# Autodesk Inventor assembly: robot
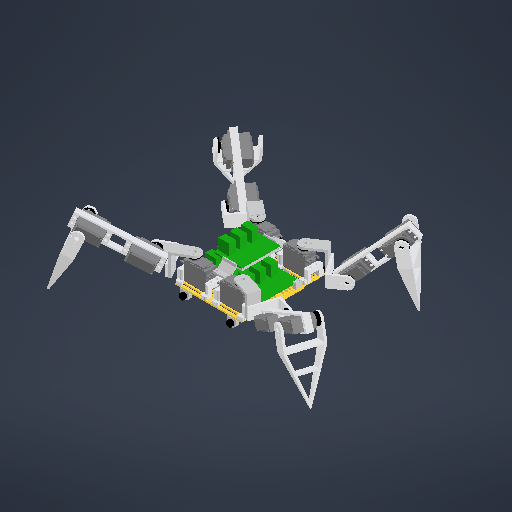
[picture p0: Inventor's stored thumbnail of the model, 512x512]
Saved by Autodesk Inventor 2026.1 (Build 301233000, 233)
## iProperties
Created: 2025-10-02
Part Number: robot
Document SubType Name: Assembly
Designer: emanuel
Author: emanuel
## Documents named in this file (16)
- C:\Users\emanuel\UnFolder\SpiderRobo\3dmodel\robot.iam
- C:\Users\emanuel\UnFolder\SpiderRobo\3dmodel\calf.ipt
- C:\Users\emanuel\UnFolder\SpiderRobo\3dmodel\femur.ipt
- C:\Users\emanuel\UnFolder\SpiderRobo\3dmodel\L1.ipt
- C:\Users\emanuel\UnFolder\SpiderRobo\3dmodel\L2.ipt
- C:\Users\emanuel\UnFolder\SpiderRobo\3dmodel\mg996r.ipt
- C:\Users\emanuel\UnFolder\SpiderRobo\3dmodel\prototype_pcb.ipt
- C:\Users\emanuel\UnFolder\SpiderRobo\3dmodel\servo_disc.ipt
- C:\Users\emanuel\UnFolder\SpiderRobo\3dmodel\servo_support_3.ipt
- C:\Users\emanuel\UnFolder\SpiderRobo\3dmodel\pcb_support_1.ipt
- C:\Users\emanuel\UnFolder\SpiderRobo\3dmodel\pcb_support_2.ipt
- C:\Users\emanuel\UnFolder\SpiderRobo\3dmodel\pcb_support_3.ipt
- C:\Users\emanuel\UnFolder\SpiderRobo\3dmodel\pcb_support_4.ipt
- C:\Users\emanuel\UnFolder\SpiderRobo\3dmodel\yellow_base.iam
- C:\Users\emanuel\UnFolder\SpiderRobo\3dmodel\screw_support.ipt
- C:\Users\emanuel\UnFolder\SpiderRobo\3dmodel\long_screw.ipt
## Components (67 placed, 15 different names)
1. calf:1 — Mate:105, Mate:106
2. femur:1 — Mate:99, Mate:100, Mate:101, Mate:102, Mate:103, Mate:104
3. L1:1 — Mate:14, Mate:15, Mate:157, Mate:158, Mate:159
4. L2:1 — Mate:107, Mate:108, Mate:154, Mate:155, Mate:156
5. mg996r:1 — Mate:12, Mate:13, Mate:92, Mate:93, Mate:94
6. prototype_pcb:1 — Mate:61, Mate:62, Flush:10
7. servo_disc:1 — Mate:12, Mate:13, Mate:14, Mate:15
8. servo_support_3:1 — Mate:11, Flush:7, Flush:8, Mate:58, Mate:87, Mate:88
9. pcb_support_1:1 — Mate:41, Mate:42, Mate:43, Mate:52
10. pcb_support_2:1 — Mate:44, Mate:45, Mate:46, Mate:50
11. pcb_support_3:1 — Mate:53, Mate:54, Mate:55, Flush:9, Mate:61
12. pcb_support_4:1 — Mate:59, Mate:60, Flush:9, Flush:10
13. yellow_base:1 [sub-assembly] — Mate:5, Mate:6, Mate:7, Mate:10, Flush:5, Flush:6, Mate:11, Flush:7, Flush:8, Mate:30, Mate:31, Mate:33, Mate:34, Mate:35, Mate:36, Mate:47, Mate:48, Mate:49, Mate:63, Mate:64, Mate:65, Mate:69, Mate:70, Mate:71, Mate:72, Mate:73, Mate:74, Mate:86, Mate:89
14. servo_support_3:2 — Mate:9, Flush:3, Flush:4, Mate:21, Mate:22
15. servo_support_3:3 — Mate:8, Flush:1, Flush:2, Mate:54, Mate:93, Mate:94
16. yellow_base:2 [sub-assembly] — Mate:2, Mate:3, Mate:4, Mate:5, Mate:6, Mate:7
17. yellow_base:3 [sub-assembly] — Mate:2, Mate:3, Mate:4, Mate:8, Flush:1, Flush:2, Mate:9, Flush:3, Flush:4, Mate:20, Mate:29, Mate:32, Mate:37, Mate:38, Mate:39, Mate:40, Mate:41, Mate:42, Mate:43, Mate:44, Mate:45, Mate:46, Mate:66, Mate:67, Mate:68, Mate:92
18. servo_support_3:4 — Mate:10, Flush:5, Flush:6, Mate:57, Mate:90, Mate:91
19. L1:2 — Mate:160, Mate:161, Mate:162
20. mg996r:2 — Mate:20, Mate:21, Mate:22, Mate:53, Mate:55, Mate:56
21. servo_disc:2
22. screw_support:1 — Mate:23, Mate:25, Mate:30, Mate:35, Mate:36
23. long_screw:1 — Mate:23, Mate:24, Mate:25
24. screw_support:2 — Mate:24, Mate:29, Mate:37
25. screw_support:3 — Mate:31, Mate:33, Mate:34
26. long_screw:2
27. screw_support:4 — Mate:32
28. pcb_support_2:2 — Mate:47, Mate:48, Mate:49, Mate:51
29. pcb_support_1:5 — Mate:38, Mate:39, Mate:40
30. prototype_pcb:2 — Mate:50, Mate:51, Mate:52
31. pcb_support_3:2 — Mate:56, Mate:57, Mate:58, Mate:59, Mate:60, Mate:62
32. pcb_support_1:6 — Mate:72, Mate:73, Mate:74, Mate:75
33. pcb_support_2:3 — Mate:63, Mate:64, Mate:65
34. pcb_support_1:7 — Mate:69, Mate:70, Mate:71, Mate:77
35. pcb_support_2:4 — Mate:66, Mate:67, Mate:68, Mate:76
36. prototype_pcb:3 — Mate:75, Mate:76, Mate:77
37. L1:3 — Mate:154, Mate:155, Mate:156
38. mg996r:3 — Mate:86, Mate:87, Mate:88
39. servo_disc:3
40. L1:4 — Mate:151, Mate:152, Mate:153
41. mg996r:4 — Mate:89, Mate:90, Mate:91
42. servo_disc:4
43. servo_disc:5 — Mate:95, Mate:96, Mate:107
44. mg996r:5 — Mate:95, Mate:96, Mate:99, Mate:100, Mate:101, Mate:108
45. servo_disc:6 — Mate:105, Mate:106
46. mg996r:6 — Mate:102, Mate:103, Mate:104
47. calf:2
48. femur:2
49. L2:2 — Mate:160, Mate:161, Mate:162
50. servo_disc:7
51. mg996r:7
52. servo_disc:8
53. mg996r:8
54. calf:3
55. femur:3
56. L2:3 — Mate:157, Mate:158, Mate:159
57. servo_disc:9
58. mg996r:9
59. servo_disc:10
60. mg996r:10
61. calf:4
62. femur:4
63. L2:4 — Mate:151, Mate:152, Mate:153
64. servo_disc:11
65. mg996r:11
66. servo_disc:12
67. mg996r:12
## Relationships (171: Mate 161, Flush 10)
- Mate:2: yellow_base:2 ↔ yellow_base:3
- Mate:3: yellow_base:2 ↔ yellow_base:3
- Mate:4: yellow_base:2 ↔ yellow_base:3
- Mate:5: yellow_base:1 ↔ yellow_base:2
- Mate:6: yellow_base:1 ↔ yellow_base:2
- Mate:7: yellow_base:1 ↔ yellow_base:2
- Mate:8: servo_support_3:3 ↔ yellow_base:3
- Flush:1: servo_support_3:3 ↔ yellow_base:3
- Flush:2: servo_support_3:3 ↔ yellow_base:3
- Mate:9: servo_support_3:2 ↔ yellow_base:3
- Flush:3: servo_support_3:2 ↔ yellow_base:3
- Flush:4: servo_support_3:2 ↔ yellow_base:3
- Mate:10: yellow_base:1 ↔ servo_support_3:4
- Flush:5: yellow_base:1 ↔ servo_support_3:4
- Flush:6: yellow_base:1 ↔ servo_support_3:4
- Mate:11: servo_support_3:1 ↔ yellow_base:1
- Flush:7: servo_support_3:1 ↔ yellow_base:1
- Flush:8: servo_support_3:1 ↔ yellow_base:1
- Mate:12: mg996r:1 ↔ servo_disc:1
- Mate:13: mg996r:1 ↔ servo_disc:1
- Mate:14: L1:1 ↔ servo_disc:1
- Mate:15: L1:1 ↔ servo_disc:1
- [Mate]: mg996r:2 ↔ servo_disc:2
- [Mate]: mg996r:2 ↔ servo_disc:2
- [Mate]: L1:2 ↔ servo_disc:2
- [Mate]: L1:2 ↔ servo_disc:2
- Mate:20: yellow_base:3 ↔ mg996r:2
- Mate:21: servo_support_3:2 ↔ mg996r:2
- Mate:22: servo_support_3:2 ↔ mg996r:2
- Mate:23: screw_support:1 ↔ long_screw:1
- Mate:24: long_screw:1 ↔ screw_support:2
- Mate:25: screw_support:1 ↔ long_screw:1
- [Mate]: screw_support:3 ↔ long_screw:2
- [Mate]: long_screw:2 ↔ screw_support:4
- [Mate]: screw_support:3 ↔ long_screw:2
- Mate:29: yellow_base:3 ↔ screw_support:2
- Mate:30: yellow_base:1 ↔ screw_support:1
- Mate:31: yellow_base:1 ↔ screw_support:3
- Mate:32: yellow_base:3 ↔ screw_support:4
- Mate:33: yellow_base:1 ↔ screw_support:3
- Mate:34: yellow_base:1 ↔ screw_support:3
- Mate:35: yellow_base:1 ↔ screw_support:1
- Mate:36: yellow_base:1 ↔ screw_support:1
- Mate:37: yellow_base:3 ↔ screw_support:2
- Mate:38: yellow_base:3 ↔ pcb_support_1:5
- Mate:39: yellow_base:3 ↔ pcb_support_1:5
- Mate:40: yellow_base:3 ↔ pcb_support_1:5
- Mate:41: pcb_support_1:1 ↔ yellow_base:3
- Mate:42: pcb_support_1:1 ↔ yellow_base:3
- Mate:43: pcb_support_1:1 ↔ yellow_base:3
- Mate:44: pcb_support_2:1 ↔ yellow_base:3
- Mate:45: pcb_support_2:1 ↔ yellow_base:3
- Mate:46: pcb_support_2:1 ↔ yellow_base:3
- Mate:47: yellow_base:1 ↔ pcb_support_2:2
- Mate:48: yellow_base:1 ↔ pcb_support_2:2
- Mate:49: yellow_base:1 ↔ pcb_support_2:2
- Mate:50: pcb_support_2:1 ↔ prototype_pcb:2
- Mate:51: pcb_support_2:2 ↔ prototype_pcb:2
- Mate:52: pcb_support_1:1 ↔ prototype_pcb:2
- Mate:53: pcb_support_3:1 ↔ mg996r:2
- Mate:54: pcb_support_3:1 ↔ servo_support_3:3
- Mate:55: pcb_support_3:1 ↔ mg996r:2
- Mate:56: mg996r:2 ↔ pcb_support_3:2
- Mate:57: servo_support_3:4 ↔ pcb_support_3:2
- Mate:58: servo_support_3:1 ↔ pcb_support_3:2
- Mate:59: pcb_support_4:1 ↔ pcb_support_3:2
- Mate:60: pcb_support_4:1 ↔ pcb_support_3:2
- Flush:9: pcb_support_3:1 ↔ pcb_support_4:1
- Mate:61: prototype_pcb:1 ↔ pcb_support_3:1
- Mate:62: prototype_pcb:1 ↔ pcb_support_3:2
- Flush:10: prototype_pcb:1 ↔ pcb_support_4:1
- Mate:63: yellow_base:1 ↔ pcb_support_2:3
- Mate:64: yellow_base:1 ↔ pcb_support_2:3
- Mate:65: yellow_base:1 ↔ pcb_support_2:3
- Mate:66: yellow_base:3 ↔ pcb_support_2:4
- Mate:67: yellow_base:3 ↔ pcb_support_2:4
- Mate:68: yellow_base:3 ↔ pcb_support_2:4
- Mate:69: yellow_base:1 ↔ pcb_support_1:7
- Mate:70: yellow_base:1 ↔ pcb_support_1:7
- Mate:71: yellow_base:1 ↔ pcb_support_1:7
- Mate:72: yellow_base:1 ↔ pcb_support_1:6
- Mate:73: yellow_base:1 ↔ pcb_support_1:6
- Mate:74: yellow_base:1 ↔ pcb_support_1:6
- Mate:75: pcb_support_1:6 ↔ prototype_pcb:3
- Mate:76: pcb_support_2:4 ↔ prototype_pcb:3
- Mate:77: pcb_support_1:7 ↔ prototype_pcb:3
- [Mate]: mg996r:3 ↔ servo_disc:3
- [Mate]: mg996r:3 ↔ servo_disc:3
- [Mate]: L1:3 ↔ servo_disc:3
- [Mate]: L1:3 ↔ servo_disc:3
- [Mate]: mg996r:4 ↔ servo_disc:4
- [Mate]: mg996r:4 ↔ servo_disc:4
- [Mate]: L1:4 ↔ servo_disc:4
- [Mate]: L1:4 ↔ servo_disc:4
- Mate:86: yellow_base:1 ↔ mg996r:3
- Mate:87: servo_support_3:1 ↔ mg996r:3
- Mate:88: servo_support_3:1 ↔ mg996r:3
- Mate:89: yellow_base:1 ↔ mg996r:4
- Mate:90: servo_support_3:4 ↔ mg996r:4
- Mate:91: servo_support_3:4 ↔ mg996r:4
- Mate:92: mg996r:1 ↔ yellow_base:3
- Mate:93: mg996r:1 ↔ servo_support_3:3
- Mate:94: mg996r:1 ↔ servo_support_3:3
- Mate:95: servo_disc:5 ↔ mg996r:5
- Mate:96: servo_disc:5 ↔ mg996r:5
- [Mate]: servo_disc:6 ↔ mg996r:6
- [Mate]: servo_disc:6 ↔ mg996r:6
- Mate:99: femur:1 ↔ mg996r:5
- Mate:100: femur:1 ↔ mg996r:5
- Mate:101: femur:1 ↔ mg996r:5
- Mate:102: femur:1 ↔ mg996r:6
- Mate:103: femur:1 ↔ mg996r:6
- Mate:104: femur:1 ↔ mg996r:6
- Mate:105: calf:1 ↔ servo_disc:6
- Mate:106: calf:1 ↔ servo_disc:6
- Mate:107: L2:1 ↔ servo_disc:5
- Mate:108: L2:1 ↔ mg996r:5
- [Mate]: servo_disc:7 ↔ mg996r:7
- [Mate]: servo_disc:7 ↔ mg996r:7
- [Mate]: servo_disc:8 ↔ mg996r:8
- [Mate]: servo_disc:8 ↔ mg996r:8
- [Mate]: femur:2 ↔ mg996r:7
- [Mate]: femur:2 ↔ mg996r:7
- [Mate]: femur:2 ↔ mg996r:7
- [Mate]: femur:2 ↔ mg996r:8
- [Mate]: femur:2 ↔ mg996r:8
- [Mate]: femur:2 ↔ mg996r:8
- [Mate]: calf:2 ↔ servo_disc:8
- [Mate]: calf:2 ↔ servo_disc:8
- [Mate]: L2:2 ↔ servo_disc:7
- [Mate]: L2:2 ↔ mg996r:7
- [Mate]: servo_disc:9 ↔ mg996r:9
- [Mate]: servo_disc:9 ↔ mg996r:9
- [Mate]: servo_disc:10 ↔ mg996r:10
- [Mate]: servo_disc:10 ↔ mg996r:10
- [Mate]: femur:3 ↔ mg996r:9
- [Mate]: femur:3 ↔ mg996r:9
- [Mate]: femur:3 ↔ mg996r:9
- [Mate]: femur:3 ↔ mg996r:10
- [Mate]: femur:3 ↔ mg996r:10
- [Mate]: femur:3 ↔ mg996r:10
- [Mate]: calf:3 ↔ servo_disc:10
- [Mate]: calf:3 ↔ servo_disc:10
- [Mate]: L2:3 ↔ servo_disc:9
- [Mate]: L2:3 ↔ mg996r:9
- [Mate]: servo_disc:11 ↔ mg996r:11
- [Mate]: servo_disc:11 ↔ mg996r:11
- [Mate]: servo_disc:12 ↔ mg996r:12
- [Mate]: servo_disc:12 ↔ mg996r:12
- [Mate]: femur:4 ↔ mg996r:11
- [Mate]: femur:4 ↔ mg996r:11
- [Mate]: femur:4 ↔ mg996r:11
- [Mate]: femur:4 ↔ mg996r:12
- [Mate]: femur:4 ↔ mg996r:12
- [Mate]: femur:4 ↔ mg996r:12
- [Mate]: calf:4 ↔ servo_disc:12
- [Mate]: calf:4 ↔ servo_disc:12
- [Mate]: L2:4 ↔ servo_disc:11
- [Mate]: L2:4 ↔ mg996r:11
- Mate:151: L1:4 ↔ L2:4
- Mate:152: L1:4 ↔ L2:4
- Mate:153: L1:4 ↔ L2:4
- Mate:154: L2:1 ↔ L1:3
- Mate:155: L2:1 ↔ L1:3
- Mate:156: L2:1 ↔ L1:3
- Mate:157: L1:1 ↔ L2:3
- Mate:158: L1:1 ↔ L2:3
- Mate:159: L1:1 ↔ L2:3
- Mate:160: L1:2 ↔ L2:2
- Mate:161: L1:2 ↔ L2:2
- Mate:162: L1:2 ↔ L2:2
## Named parameters: d25_d21 = 0 mm, d26_d22 = 0 mm, d27_d23 = 0 mm, d28_d24 = 0 mm, d35_d32 = 0 mm, d36_d33 = 0 mm, d37_d34 = 0 mm, d95_d21 = 0 mm, d96_d22 = 0 mm, d97_d23 = 0 mm, d98_d24 = 0 mm, d99_d21 = 0 mm, d100_d22 = 0 mm, d101_d23 = 0 mm, d102_d24 = 0 mm, d114_d112 = 0 mm, d115_d113 = 0 mm, d126_d112 = 0 mm, d127_d113 = 0 mm, d128_d114_d112 = 0 mm, d129_d115_d113 = 0 mm, d130_d116 = 0 mm, d131_d117 = 0 mm, d132_d118 = 0 mm, d133_d119 = 0 mm, d134_d120 = 0 mm, d135_d121 = 0 mm, d136_d122 = 0 mm, d137_d123 = 0 mm, d138_d124 = 0 mm, d139_d125 = 0 mm, d140_d112 = 0 mm, d141_d113 = 0 mm, d142_d114_d112 = 0 mm, d143_d115_d113 = 0 mm, d144_d116 = 0 mm, d145_d117 = 0 mm, d146_d118 = 0 mm, d147_d119 = 0 mm, d148_d120 = 0 mm, d149_d121 = 0 mm, d150_d122 = 0 mm, d151_d123 = 0 mm, d152_d124 = 0 mm, d153_d125 = 0 mm, d154_d112 = 0 mm, d155_d113 = 0 mm, d156_d114_d112 = 0 mm, d157_d115_d113 = 0 mm, d158_d116 = 0 mm, d159_d117 = 0 mm, d160_d118 = 0 mm, d161_d119 = 0 mm, d162_d120 = 0 mm, d163_d121 = 0 mm, d164_d122 = 0 mm, d165_d123 = 0 mm, d166_d124 = 0 mm, d167_d125 = 0 mm
